# Autodesk Inventor assembly: BikeAssembly
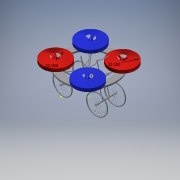
[picture p0: Inventor's stored thumbnail of the model, 180x180]
Saved by Autodesk Inventor 2019 (Build 230136000, 136)
## iProperties
Created: 2020-01-15
Part Number: BikeAssembly
Document SubType Name: Assembly
Designer: 18186
Author: 18186
## Documents named in this file (11)
- D:\Bike\BikeAssembly.iam
- D:\Bike\Bike Frame.ipt
- D:\Bike\Bearing.ipt
- D:\Bike\Fork.ipt
- D:\Bike\Axle.ipt
- D:\Bike\Nut.ipt
- D:\Bike\Bike Wheel.ipt
- D:\Bike\Propeller Motor Guard Assembly CCW.iam
- D:\Bike\Propeller Bolt.ipt
- D:\Bike\Propeller Motor Guard Assembly CW.iam
- D:\Bike\PropellorGuardTop.ipt
## Components (58 placed, 10 different names)
1. Bike Frame:1 — Insert:4, Mate:1, Flush:1, Mate:2, Mate:3, Mate:4, Flush:2, Mate:5, Flush:3, Flush:4, Flush:5, Mate:6, Mate:7, Mate:45, Mate:46, Mate:47, Mate:48, Insert:5, Mate:49, Insert:15, Mate:52, Insert:16, Mate:53
2. Bearing:3 — Insert:4, Flush:5, Mate:7
3. Bearing:4 — Mate:1, Flush:1, Flush:4, Mate:6
4. Fork:1 — Mate:2, Mate:3, Mate:41, Flush:14, Mate:42, Flush:15
5. Bearing:5 — Mate:41, Flush:14, Mate:43
6. Bearing:6 — Mate:8, Flush:15, Mate:44
7. Bearing:7 — Mate:5, Flush:3, Mate:9, Mate:15
8. Bearing:8 — Mate:4, Flush:2, Mate:17
9. Axle:1 — Mate:8, Mate:10, Mate:12, Mate:26, Mate:28, Mate:34, Mate:36, Mate:42
10. Axle:2 — Mate:9, Mate:14, Mate:16, Mate:30, Mate:32, Mate:37, Mate:39
11. Nut:1 — Mate:16, Mate:17, Mate:33
12. Nut:2 — Mate:14, Mate:15, Mate:31
13. Nut:3 — Mate:10, Mate:27, Mate:44
14. Nut:4 — Mate:12, Mate:29, Mate:43
15. Bike Wheel:1 — Mate:18, Flush:6, Mate:19, Flush:7
16. Bearing:9 — Mate:18, Flush:6
17. Bearing:10 — Mate:19, Flush:7, Mate:26, Mate:27
18. Bike Wheel:2
19. Bearing:11 — Mate:29
20. Bearing:12 — Mate:28, Mate:35
21. Bike Wheel:3
22. Bearing:13 — Mate:31
23. Bearing:14 — Mate:30, Mate:40
24. Bike Wheel:4
25. Bearing:15 — Mate:38
26. Bearing:16 — Mate:32, Mate:33
27. Nut:5 — Mate:37, Mate:38
28. Nut:6 — Mate:39, Mate:40
29. Nut:7 — Mate:36
30. Nut:8 — Mate:34, Mate:35
31. Propeller Motor Guard Assembly CCW:1 [sub-assembly] — Mate:45, Mate:46, Mate:47, Mate:48, Insert:10, Insert:11, Insert:12, Insert:13, Insert:14, Mate:58, Mate:59
32. Propeller Motor Guard Assembly CCW:3 [sub-assembly] — Insert:5, Mate:49, Mate:50, Mate:51, Insert:6, Insert:7, Insert:8, Insert:9, Mate:56, Mate:57
33. Propeller Bolt:1 — Insert:6
34. Propeller Bolt:2 — Insert:9
35. Propeller Bolt:3 — Insert:7
36. Propeller Bolt:4 — Insert:8
37. Propeller Bolt:5 — Mate:50, Mate:51
38. Propeller Bolt:6 — Insert:14
39. Propeller Bolt:7 — Insert:12
40. Propeller Bolt:8 — Insert:13
41. Propeller Bolt:9 — Insert:11
42. Propeller Bolt:10 — Insert:10
43. Propeller Motor Guard Assembly CW:1 [sub-assembly] — Insert:16, Mate:53, Insert:17, Insert:18, Insert:19, Insert:20, Insert:21, Mate:60, Mate:61
44. Propeller Motor Guard Assembly CW:2 [sub-assembly] — Insert:15, Mate:52, Insert:22, Insert:23, Insert:24, Insert:25, Insert:26, Mate:54, Mate:55
45. Propeller Bolt:11 — Insert:18
46. Propeller Bolt:12 — Insert:19
47. Propeller Bolt:13 — Insert:20
48. Propeller Bolt:14 — Insert:17
49. Propeller Bolt:15 — Insert:21
50. Propeller Bolt:16 — Insert:24
51. Propeller Bolt:17 — Insert:23
52. Propeller Bolt:18 — Insert:26
53. Propeller Bolt:19 — Insert:25
54. Propeller Bolt:20 — Insert:22
55. PropellorGuardTop:1 — Mate:56, Mate:57
56. PropellorGuardTop:2 — Mate:58, Mate:59
57. PropellorGuardTop:3 — Mate:54, Mate:55
58. PropellorGuardTop:4 — Mate:60, Mate:61
## Relationships (97: Mate 59, Insert 23, Flush 15)
- Insert:4: Bike Frame:1 ↔ Bearing:3
- Mate:1: Bike Frame:1 ↔ Bearing:4
- Flush:1: Bike Frame:1 ↔ Bearing:4
- Mate:2: Bike Frame:1 ↔ Fork:1
- Mate:3: Bike Frame:1 ↔ Fork:1
- Mate:4: Bike Frame:1 ↔ Bearing:8
- Flush:2: Bike Frame:1 ↔ Bearing:8
- Mate:5: Bike Frame:1 ↔ Bearing:7
- Flush:3: Bike Frame:1 ↔ Bearing:7
- Flush:4: Bike Frame:1 ↔ Bearing:4
- Flush:5: Bike Frame:1 ↔ Bearing:3
- Mate:6: Bike Frame:1 ↔ Bearing:4
- Mate:7: Bike Frame:1 ↔ Bearing:3
- Mate:8: Bearing:6 ↔ Axle:1
- Mate:9: Bearing:7 ↔ Axle:2
- Mate:10: Axle:1 ↔ Nut:3
- Mate:12: Axle:1 ↔ Nut:4
- Mate:14: Axle:2 ↔ Nut:2
- Mate:15: Bearing:7 ↔ Nut:2
- Mate:16: Axle:2 ↔ Nut:1
- Mate:17: Bearing:8 ↔ Nut:1
- Mate:18: Bike Wheel:1 ↔ Bearing:9
- Flush:6: Bike Wheel:1 ↔ Bearing:9
- Mate:19: Bike Wheel:1 ↔ Bearing:10
- Flush:7: Bike Wheel:1 ↔ Bearing:10
- [Mate]: Bike Wheel:2 ↔ Bearing:11
- [Flush]: Bike Wheel:2 ↔ Bearing:11
- [Mate]: Bike Wheel:2 ↔ Bearing:12
- [Flush]: Bike Wheel:2 ↔ Bearing:12
- [Mate]: Bike Wheel:3 ↔ Bearing:13
- [Flush]: Bike Wheel:3 ↔ Bearing:13
- [Mate]: Bike Wheel:3 ↔ Bearing:14
- [Flush]: Bike Wheel:3 ↔ Bearing:14
- [Mate]: Bike Wheel:4 ↔ Bearing:15
- [Flush]: Bike Wheel:4 ↔ Bearing:15
- [Mate]: Bike Wheel:4 ↔ Bearing:16
- [Flush]: Bike Wheel:4 ↔ Bearing:16
- Mate:26: Axle:1 ↔ Bearing:10
- Mate:27: Nut:3 ↔ Bearing:10
- Mate:28: Axle:1 ↔ Bearing:12
- Mate:29: Nut:4 ↔ Bearing:11
- Mate:30: Axle:2 ↔ Bearing:14
- Mate:31: Nut:2 ↔ Bearing:13
- Mate:32: Axle:2 ↔ Bearing:16
- Mate:33: Nut:1 ↔ Bearing:16
- Mate:34: Axle:1 ↔ Nut:8
- Mate:35: Bearing:12 ↔ Nut:8
- Mate:36: Axle:1 ↔ Nut:7
- Mate:37: Axle:2 ↔ Nut:5
- Mate:38: Bearing:15 ↔ Nut:5
- Mate:39: Axle:2 ↔ Nut:6
- Mate:40: Bearing:14 ↔ Nut:6
- Mate:41: Fork:1 ↔ Bearing:5
- Flush:14: Fork:1 ↔ Bearing:5
- Mate:42: Fork:1 ↔ Axle:1
- Flush:15: Fork:1 ↔ Bearing:6
- Mate:43: Bearing:5 ↔ Nut:4
- Mate:44: Bearing:6 ↔ Nut:3
- Mate:45: Bike Frame:1 ↔ Propeller Motor Guard Assembly CCW:1
- Mate:46: Bike Frame:1 ↔ Propeller Motor Guard Assembly CCW:1
- Mate:47: Bike Frame:1 ↔ Propeller Motor Guard Assembly CCW:1
- Mate:48: Bike Frame:1 ↔ Propeller Motor Guard Assembly CCW:1
- Insert:5: Bike Frame:1 ↔ Propeller Motor Guard Assembly CCW:3
- Mate:49: Bike Frame:1 ↔ Propeller Motor Guard Assembly CCW:3
- Mate:50: Propeller Motor Guard Assembly CCW:3 ↔ Propeller Bolt:5
- Mate:51: Propeller Motor Guard Assembly CCW:3 ↔ Propeller Bolt:5
- Insert:6: Propeller Motor Guard Assembly CCW:3 ↔ Propeller Bolt:1
- Insert:7: Propeller Motor Guard Assembly CCW:3 ↔ Propeller Bolt:3
- Insert:8: Propeller Motor Guard Assembly CCW:3 ↔ Propeller Bolt:4
- Insert:9: Propeller Motor Guard Assembly CCW:3 ↔ Propeller Bolt:2
- Insert:10: Propeller Motor Guard Assembly CCW:1 ↔ Propeller Bolt:10
- Insert:11: Propeller Motor Guard Assembly CCW:1 ↔ Propeller Bolt:9
- Insert:12: Propeller Motor Guard Assembly CCW:1 ↔ Propeller Bolt:7
- Insert:13: Propeller Motor Guard Assembly CCW:1 ↔ Propeller Bolt:8
- Insert:14: Propeller Motor Guard Assembly CCW:1 ↔ Propeller Bolt:6
- Insert:15: Bike Frame:1 ↔ Propeller Motor Guard Assembly CW:2
- Mate:52: Bike Frame:1 ↔ Propeller Motor Guard Assembly CW:2
- Insert:16: Bike Frame:1 ↔ Propeller Motor Guard Assembly CW:1
- Mate:53: Bike Frame:1 ↔ Propeller Motor Guard Assembly CW:1
- Insert:17: Propeller Motor Guard Assembly CW:1 ↔ Propeller Bolt:14
- Insert:18: Propeller Motor Guard Assembly CW:1 ↔ Propeller Bolt:11
- Insert:19: Propeller Motor Guard Assembly CW:1 ↔ Propeller Bolt:12
- Insert:20: Propeller Motor Guard Assembly CW:1 ↔ Propeller Bolt:13
- Insert:21: Propeller Motor Guard Assembly CW:1 ↔ Propeller Bolt:15
- Insert:22: Propeller Motor Guard Assembly CW:2 ↔ Propeller Bolt:20
- Insert:23: Propeller Motor Guard Assembly CW:2 ↔ Propeller Bolt:17
- Insert:24: Propeller Motor Guard Assembly CW:2 ↔ Propeller Bolt:16
- Insert:25: Propeller Motor Guard Assembly CW:2 ↔ Propeller Bolt:19
- Insert:26: Propeller Motor Guard Assembly CW:2 ↔ Propeller Bolt:18
- Mate:54: Propeller Motor Guard Assembly CW:2 ↔ PropellorGuardTop:3
- Mate:55: Propeller Motor Guard Assembly CW:2 ↔ PropellorGuardTop:3
- Mate:56: Propeller Motor Guard Assembly CCW:3 ↔ PropellorGuardTop:1
- Mate:57: Propeller Motor Guard Assembly CCW:3 ↔ PropellorGuardTop:1
- Mate:58: Propeller Motor Guard Assembly CCW:1 ↔ PropellorGuardTop:2
- Mate:59: Propeller Motor Guard Assembly CCW:1 ↔ PropellorGuardTop:2
- Mate:60: Propeller Motor Guard Assembly CW:1 ↔ PropellorGuardTop:4
- Mate:61: Propeller Motor Guard Assembly CW:1 ↔ PropellorGuardTop:4
## Named parameters: d32_d28 = 0 mm, d33_d29 = 0 mm, d34_d30 = 0 mm, d35_d31 = 0 mm, d36_d28 = 0 mm, d37_d29 = 0 mm, d38_d30 = 0 mm, d39_d31 = 0 mm, d40_d28 = 0 mm, d41_d29 = 0 mm, d42_d30 = 0 mm, d43_d31 = 0 mm
